# Autodesk Inventor assembly: X02598_LEGOmini_LowerBody
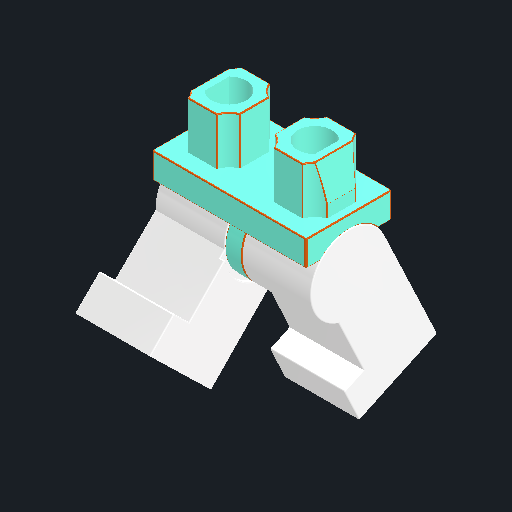
[picture p0: Inventor's stored thumbnail of the model, 512x512]
Saved by Autodesk Inventor 2022 (Build 260153000, 153)
## iProperties
Created: 2022-02-05
Part Number: X02598_LEGOmini_LowerBody
Document SubType Name: Assembly
Designer: Jason
Author: Jason
## Documents named in this file (4)
- D:\D-disk\pomelo\大一\下學期\機械設計製圖\110033226_LEGOmini\110033226_LEGOmini_天使\110033226_LEGOmini_天使下半身.iam
- D:\D-disk\pomelo\大一\下學期\機械設計製圖\110033226_LEGOmini\110033226_LEGOmini_天使\110033226_LEGOmini_天使腰部.ipt
- D:\D-disk\pomelo\大一\下學期\機械設計製圖\110033226_LEGOmini\110033226_LEGOmini_天使\110033226_LEGOmini_天使右腳.ipt
- D:\D-disk\pomelo\大一\下學期\機械設計製圖\110033226_LEGOmini\110033226_LEGOmini_天使\110033226_LEGOmini_天使左腳.ipt
## Components (3 placed, 3 different names)
1. 110033226_LEGOmini_天使腰部:1 — 插入:1, 插入:2
2. 110033226_LEGOmini_天使右腳:1 — 插入:1
3. 110033226_LEGOmini_天使左腳:1 — 插入:2
## Relationships (2: Insert 2)
- 插入:1 [Insert]: 110033226_LEGOmini_天使腰部:1 ↔ 110033226_LEGOmini_天使右腳:1
- 插入:2 [Insert]: 110033226_LEGOmini_天使腰部:1 ↔ 110033226_LEGOmini_天使左腳:1
